# Autodesk Inventor assembly: frontChassisAssembly
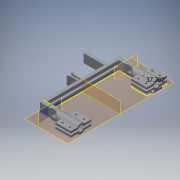
[picture p0: Inventor's stored thumbnail of the model, 180x180]
Saved by Autodesk Inventor 2018 (Build 220112000, 112)
## iProperties
Created: 2017-10-04
Part Number: frontChassisAssembly
Document SubType Name: Assembly
Designer: Payal Jindal
Author: Payal Jindal
## Documents named in this file (3)
- C:\Users\Payal Jindal\Documents\Inventor\Mousetrap\frontChassisAssembly.iam
- C:\Users\Payal Jindal\Documents\Inventor\Mousetrap\frontChassis.ipt
- C:\Users\Payal Jindal\Documents\Inventor\Mousetrap\frontChassisMirror.ipt
## Components (2 placed, 2 different names)
1. frontChassis:1 — Mate:1, Flush:1, Flush:2
2. frontChassisMirror:1 — Mate:1, Flush:1, Flush:2
## Relationships (3: Flush 2, Mate 1)
- Mate:1: frontChassis:1 ↔ frontChassisMirror:1
- Flush:1: frontChassis:1 ↔ frontChassisMirror:1
- Flush:2: frontChassis:1 ↔ frontChassisMirror:1
